# Autodesk Inventor assembly: МПСТ Редуктор
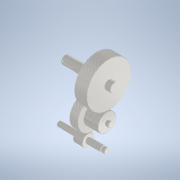
[picture p0: Inventor's stored thumbnail of the model, 180x180]
Saved by Autodesk Inventor 2022 (Build 260153070, 153G)
## iProperties
Created: 2021-09-16
Part Number: МПСТ Редуктор
Document SubType Name: Assembly
Designer: Алексанян Г.
Author: Алексанян Г.
## Documents named in this file (6)
- C:\Users\Гарник\Desktop\учёба\5 семак\Детмаш\Reductor\МПСТ Редуктор.iam
- C:\Users\Гарник\Desktop\учёба\5 семак\Детмаш\Reductor\МПСТ Промежуточный Вал.iam
- C:\Users\Гарник\Desktop\учёба\5 семак\Детмаш\Reductor\МПСТ Тихоходный Вал.iam
- C:\Users\Гарник\Desktop\учёба\5 семак\Детмаш\Reductor\МПСТ Редуктор\Мастер проектирования\Цилиндрическое зубчатое зацепление1.iam
- C:\Users\Гарник\Desktop\учёба\5 семак\Детмаш\Reductor\МПСТ Быстроходный Вал.iam
- C:\Users\Гарник\Desktop\учёба\5 семак\Детмаш\Reductor\МПСТ Редуктор\Мастер проектирования\Цилиндрическое зубчатое зацепление2.iam
## Components (5 placed, 4 different names)
1. МПСТ Промежуточный Вал:1 [sub-assembly] — Угол:1, Совмещение:1, Совмещение:2, Заподлицо:1, Совмещение:5, Совмещение:7, Совмещение:8
2. МПСТ Тихоходный Вал:1 [sub-assembly] — Угол:1, Совмещение:1, Совмещение:3, Совмещение:4
3. Цилиндрическое зубчатое зацепление:1 [sub-assembly] — Совмещение:2, Заподлицо:1, Совмещение:3, Совмещение:4
4. МПСТ Быстроходный Вал:1 [sub-assembly] — Совмещение:5, Совмещение:6, Заподлицо:2
5. Цилиндрическое зубчатое зацепление:2 [sub-assembly] — Совмещение:6, Заподлицо:2, Совмещение:7, Совмещение:8
## Relationships (11: Mate 8, Flush 2, Angle 1)
- Угол:1 [Angle] (0 deg): МПСТ Промежуточный Вал:1 ↔ МПСТ Тихоходный Вал:1
- Совмещение:1 [Mate] (300 mm): МПСТ Промежуточный Вал:1 ↔ МПСТ Тихоходный Вал:1
- Совмещение:2 [Mate]: МПСТ Промежуточный Вал:1 ↔ Цилиндрическое зубчатое зацепление:1
- Заподлицо:1 [Flush]: МПСТ Промежуточный Вал:1 ↔ Цилиндрическое зубчатое зацепление:1
- Совмещение:3 [Mate]: МПСТ Тихоходный Вал:1 ↔ Цилиндрическое зубчатое зацепление:1
- Совмещение:4 [Mate]: МПСТ Тихоходный Вал:1 ↔ Цилиндрическое зубчатое зацепление:1
- Совмещение:5 [Mate] (200 mm): МПСТ Промежуточный Вал:1 ↔ МПСТ Быстроходный Вал:1
- Совмещение:6 [Mate]: МПСТ Быстроходный Вал:1 ↔ Цилиндрическое зубчатое зацепление:2
- Заподлицо:2 [Flush]: МПСТ Быстроходный Вал:1 ↔ Цилиндрическое зубчатое зацепление:2
- Совмещение:7 [Mate]: МПСТ Промежуточный Вал:1 ↔ Цилиндрическое зубчатое зацепление:2
- Совмещение:8 [Mate]: МПСТ Промежуточный Вал:1 ↔ Цилиндрическое зубчатое зацепление:2
